# Autodesk Inventor assembly: ThighRightNCS
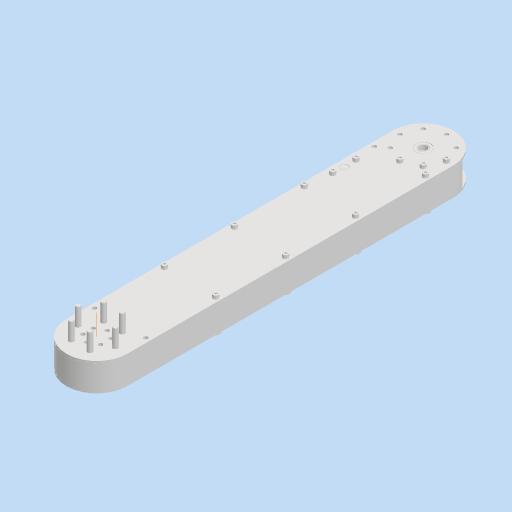
[picture p0: Inventor's stored thumbnail of the model, 512x512]
Saved by Autodesk Inventor 2023 (Build 270158000, 158)
## iProperties
Created: 2026-06-18
Part Number: ThighRightNCS
Document SubType Name: Assembly
Designer: Nathann
Author: Nathann
## Documents named in this file (2)
- C:\Users\Nathann\ClawdDrive\Objet3D\RunningRobot\PartURDF\ThighRightNCS.iam
- C:\Users\Nathann\ClawdDrive\Objet3D\RunningRobot\PartURDF\ThighRight.iam
## Components (1 placed, 1 different names)
1. ThighRight:1 [sub-assembly] — Flush:1, Mate:1, Angle:1
## Relationships (5: Mate 3, Flush 1, Angle 1)
- Flush:1: ThighRight:1
- Mate:1: ThighRight:1
- Mate:2
- Mate:3
- Angle:1 (180 deg): ThighRight:1
